# Autodesk Inventor assembly: Body Chassis Assembly
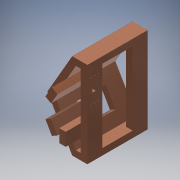
[picture p0: Inventor's stored thumbnail of the model, 180x180]
Saved by Autodesk Inventor 2017 (Build 210142000, 142)
## iProperties
Created: 2018-10-18
Part Number: Body Chassis Assembly
Document SubType Name: Assembly
Designer: Dell
Author: Dell
## Documents named in this file (6)
- C:\Users\Dell\Documents\GitHub\tr2\Body\Body Chassis Assembly.iam
- C:\Users\Dell\Documents\GitHub\tr2\Body\BO01.ipt
- C:\Users\Dell\Documents\GitHub\tr2\Body\BO02.ipt
- C:\Users\Dell\Documents\GitHub\tr2\Body\BO03.ipt
- C:\Users\Dell\Documents\GitHub\tr2\Body\BO14.ipt
- C:\Users\Dell\Documents\GitHub\tr2\Body\BO15.ipt
## Components (15 placed, 5 different names)
1. BO01:1 — Mate:15, Flush:20, Flush:21, Mate:16, Mate:23
2. BO01:2
3. BO02:1 — Mate:20, Flush:25
4. BO02:2
5. BO01:3 — Mate:21
6. BO01:4 — Mate:22
7. BO02:3 — Mate:19, Flush:26
8. BO02:4
9. BO01:5
10. BO01:6 — Flush:22, Flush:23
11. BO03:2 — Flush:22, Flush:23, Mate:16, Flush:24, Mate:17
12. BO14:1 — Mate:15, Flush:20, Flush:21
13. BO15:1 — Flush:24, Mate:17, Mate:23
14. BO15:2 — Mate:20, Flush:25, Mate:21
15. BO15:3 — Mate:19, Flush:26, Mate:22
## Relationships (42: Flush 22, Mate 20)
- [Mate]: BO01:1 ↔ BO01:2
- [Mate]: BO01:1 ↔ BO01:2
- [Flush]: BO01:1 ↔ BO01:2
- [Mate]: BO01:2 ↔ BO02:1
- [Flush]: BO01:2 ↔ BO02:1
- [Flush]: BO01:2 ↔ BO02:1
- [Mate]: BO01:2 ↔ BO02:2
- [Flush]: BO01:2 ↔ BO02:2
- [Flush]: BO01:2 ↔ BO02:2
- [Mate]: BO01:3 ↔ BO01:4
- [Mate]: BO01:3 ↔ BO01:4
- [Flush]: BO01:3 ↔ BO01:4
- [Mate]: BO01:4 ↔ BO02:3
- [Flush]: BO01:4 ↔ BO02:3
- [Flush]: BO01:4 ↔ BO02:3
- [Mate]: BO01:4 ↔ BO02:4
- [Flush]: BO01:4 ↔ BO02:4
- [Flush]: BO01:4 ↔ BO02:4
- [Mate]: BO02:1 ↔ BO01:3
- [Flush]: BO02:1 ↔ BO01:3
- [Flush]: BO02:1 ↔ BO01:3
- [Mate]: BO01:5 ↔ BO01:6
- [Mate]: BO01:5 ↔ BO01:6
- [Flush]: BO01:5 ↔ BO01:6
- [Mate]: BO02:3 ↔ BO01:5
- [Flush]: BO02:3 ↔ BO01:5
- [Flush]: BO02:3 ↔ BO01:5
- Mate:15: BO01:1 ↔ BO14:1
- Flush:20: BO01:1 ↔ BO14:1
- Flush:21: BO01:1 ↔ BO14:1
- Flush:22: BO01:6 ↔ BO03:2
- Flush:23: BO01:6 ↔ BO03:2
- Mate:16: BO01:1 ↔ BO03:2
- Flush:24: BO03:2 ↔ BO15:1
- Mate:17: BO03:2 ↔ BO15:1
- Mate:19: BO02:3 ↔ BO15:3
- Mate:20: BO02:1 ↔ BO15:2
- Flush:25: BO02:1 ↔ BO15:2
- Flush:26: BO02:3 ↔ BO15:3
- Mate:21: BO01:3 ↔ BO15:2
- Mate:22: BO01:4 ↔ BO15:3
- Mate:23 (76.2 mm): BO01:1 ↔ BO15:1
## Named parameters: d8_d30 = 0 mm, d9_d31 = 0 mm, d10_d32 = 0 mm, d12_d2 = 0 mm, d13_d3 = 0 mm, d14_d4 = 0 mm, d15_d5 = 0 mm, d16_d6 = 0 mm, d17_d7 = 0 mm, d18_d8 = 0 mm, d19_d0 = 0 mm, d20_d1 = 0 mm, d24_d2 = 0 mm, d28_d0 = 0 mm, d29_d1 = 0 mm
